# Autodesk Inventor assembly: Assem6speedgearbox
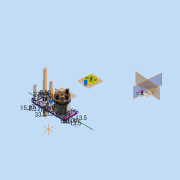
[picture p0: Inventor's stored thumbnail of the model, 180x180]
Saved by Autodesk Inventor 2022 (Build 260153000, 153)
## iProperties
Created: 2024-04-23
Part Number: Assem6speedgearbox
Document SubType Name: Assembly
Designer: ktamu
Author: ktamu
## Documents named in this file (11)
- D:\SDinventor\GearBox6Speed\Assem6speedgearbox.iam
- D:\SDinventor\GearBox6Speed\B1cover.ipt
- D:\SDinventor\GearBox6Speed\B3board.ipt
- D:\SDinventor\GearBox6Speed\driveshaft.ipt
- D:\SDinventor\GearBox6Speed\shaft4x45.ipt
- D:\SDinventor\GearBox6Speed\GearHub6kakku.ipt
- D:\SDinventor\GearBox6Speed\G9hub.ipt
- D:\SDinventor\GearBox6Speed\motor_for6speedgearbox.ipt
- D:\SDinventor\GearBox6Speed\motorshaft2x38.ipt
- D:\SDinventor\GearBox6Speed\Assem6speedgearbox\デザイン アクセラレータ\平歯車autoB1.iam
- D:\SDinventor\GearBox6Speed\Assem6speedgearbox\デザイン アクセラレータ\auto8-36g111.iam
## Components (10 placed, 10 different names)
1. B1cover:1 — 挿入:8, 回転:3
2. B3board:1 — 挿入:2, 挿入:4, メイト:1, 挿入:6, 角度:1
3. driveshaft:1 — 挿入:2, 挿入:3, 回転:1
4. shaft4x45:1 — 挿入:4, 挿入:5, 回転:2
5. GearHub6kakku:1 — 挿入:3, 回転:1
6. G9hub:1 — 挿入:5, 回転:2
7. motor_for6speedgearbox:1 — メイト:1, 挿入:6, 角度:1, 挿入:7, 挿入:8, 回転:3
8. motorshaft2x38:1 — 挿入:7
9. auto8-36g11:1 [sub-assembly] — メイト:2, フラッシュ:1
10. auto14-36g7andYell:1 [sub-assembly]
## Relationships (14: Insert 7, RelateRotation 3, Mate 2, Angle 1, Flush 1)
- 挿入:2 [Insert] (-26 mm): B3board:1 ↔ driveshaft:1
- 挿入:3 [Insert] (-46 mm): driveshaft:1 ↔ GearHub6kakku:1
- 回転:1 [RelateRotation] (1 ul): driveshaft:1 ↔ GearHub6kakku:1
- 挿入:4 [Insert] (-11.3 mm): B3board:1 ↔ shaft4x45:1
- 挿入:5 [Insert] (31 mm): shaft4x45:1 ↔ G9hub:1
- 回転:2 [RelateRotation] (1 ul): shaft4x45:1 ↔ G9hub:1
- メイト:1 [Mate]: B3board:1 ↔ motor_for6speedgearbox:1
- 挿入:6 [Insert]: B3board:1 ↔ motor_for6speedgearbox:1
- 角度:1 [Angle] (0 deg): B3board:1 ↔ motor_for6speedgearbox:1
- 挿入:7 [Insert] (-6.9 mm): motor_for6speedgearbox:1 ↔ motorshaft2x38:1
- 挿入:8 [Insert]: B1cover:1 ↔ motor_for6speedgearbox:1
- 回転:3 [RelateRotation] (1 ul): B1cover:1 ↔ motor_for6speedgearbox:1
- メイト:2 [Mate]: auto8-36g11:1
- フラッシュ:1 [Flush]: auto8-36g11:1
